# Autodesk Inventor assembly: BatteryBox
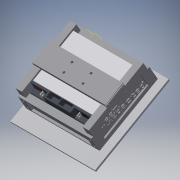
[picture p0: Inventor's stored thumbnail of the model, 180x180]
Saved by Autodesk Inventor 2016 (Build 200138000, 138)
## iProperties
Created: 2017-01-04
Part Number: BatteryBox
Document SubType Name: Assembly
Designer: james
Author: james
## Documents named in this file (8)
- C:\Users\james\Documents\Inventor\2017Ri3D\BatteryBox.iam
- C:\Users\james\Documents\Inventor\2017Ri3D\Floor.ipt
- C:\Users\james\Documents\Inventor\2017Ri3D\Battery.ipt
- C:\Users\james\Documents\Inventor\2017Ri3D\SideWall.ipt
- C:\Users\james\Documents\Inventor\2017Ri3D\BottomWall.ipt
- C:\Users\james\Documents\Inventor\2017Ri3D\TopPlate.ipt
- C:\Users\james\Documents\Inventor\2017Ri3D\BottomPlate.iam
- C:\Users\james\Documents\Inventor\2017Ri3D\sideplate.ipt
## Components (8 placed, 7 different names)
1. Floor:1 — Mate:1, Mate:15, Mate:16, Mate:17, Mate:23
2. Battery:1 — Mate:1, Mate:14, Mate:26
3. SideWall:1 — Mate:23, Mate:24, Mate:25
4. SideWall:2 — Mate:17, Mate:18, Mate:19, Mate:20, Mate:21, Mate:22, Mate:26, Flush:1, Mate:28, Mate:31, Mate:32
5. BottomWall:2 — Mate:14, Mate:15, Mate:19, Mate:20, Mate:21, Mate:25
6. TopPlate:1 — Flush:1, Mate:29, Mate:30
7. BottomPlate:1 [sub-assembly] — Mate:16, Mate:18, Mate:22, Mate:24
8. sideplate:1 — Mate:28, Mate:29, Mate:30, Mate:31, Mate:32
## Relationships (20: Mate 19, Flush 1)
- Mate:1: Floor:1 ↔ Battery:1
- Mate:14: Battery:1 ↔ BottomWall:2
- Mate:15: Floor:1 ↔ BottomWall:2
- Mate:16: Floor:1 ↔ BottomPlate:1
- Mate:17: Floor:1 ↔ SideWall:2
- Mate:18: SideWall:2 ↔ BottomPlate:1
- Mate:19: SideWall:2 ↔ BottomWall:2
- Mate:20: SideWall:2 ↔ BottomWall:2
- Mate:21: SideWall:2 ↔ BottomWall:2
- Mate:22: SideWall:2 ↔ BottomPlate:1
- Mate:23: Floor:1 ↔ SideWall:1
- Mate:24: SideWall:1 ↔ BottomPlate:1
- Mate:25: SideWall:1 ↔ BottomWall:2
- Mate:26: Battery:1 ↔ SideWall:2
- Flush:1: SideWall:2 ↔ TopPlate:1
- Mate:28: SideWall:2 ↔ sideplate:1
- Mate:29: TopPlate:1 ↔ sideplate:1
- Mate:30: TopPlate:1 ↔ sideplate:1
- Mate:31: SideWall:2 ↔ sideplate:1
- Mate:32: SideWall:2 ↔ sideplate:1
